# Autodesk Inventor assembly: NMR Frame
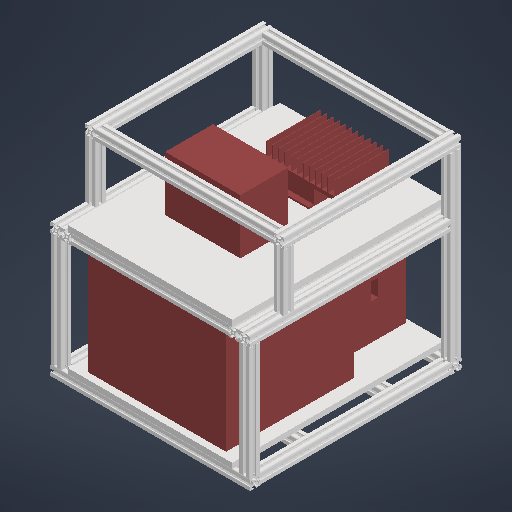
[picture p0: Inventor's stored thumbnail of the model, 512x512]
Saved by Autodesk Inventor 2026.2 (Build 302298010, 298A)
## iProperties
Created: 2026-08-09
Part Number: NMR Frame
Document SubType Name: Assembly
Designer: aiden
Author: aiden
## Documents named in this file (15)
- D:\[GitHub]\flowthrough-water-quality-monitoring-system\system_development\Moultrie\v0.4.2\NMRtray\Frame\NMR Frame.iam
- D:\[GitHub]\flowthrough-water-quality-monitoring-system\system_development\Moultrie\v0.4.2\NMRtray\Al Bars\AL369.575_5537T104.ipt
- D:\[GitHub]\flowthrough-water-quality-monitoring-system\system_development\Moultrie\v0.4.2\NMRtray\Al Bars\AL210_5537T104.ipt
- D:\[GitHub]\flowthrough-water-quality-monitoring-system\system_development\Moultrie\v0.4.2\NMRtray\Al Bars\AL336_5537T104.ipt
- D:\[GitHub]\flowthrough-water-quality-monitoring-system\system_development\Moultrie\v0.4.2\NMRtray\Al Bars\AL329.575_5537T104.ipt
- D:\[GitHub]\flowthrough-water-quality-monitoring-system\system_development\Moultrie\v0.4.2\NMRtray\Al Bars\AL106_5537T104.ipt
- D:\[GitHub]\flowthrough-water-quality-monitoring-system\system_development\Moultrie\v0.4.2\NMRtray\Al Bars\AL373.7_5537T104.ipt
- D:\[GitHub]\flowthrough-water-quality-monitoring-system\system_development\Moultrie\v0.4.2\NMRtray\Al Bars\AL393.7_5537T104.ipt
- D:\[GitHub]\flowthrough-water-quality-monitoring-system\system_development\Moultrie\v0.4.2\NMRtray\Al Bars\AL289.575_5537T104.ipt
- D:\[GitHub]\flowthrough-water-quality-monitoring-system\system_development\Moultrie\v0.4.2\NMRtray\Shelf.ipt
- D:\[GitHub]\flowthrough-water-quality-monitoring-system\system_development\Moultrie\v0.4.2\NMRtray\Electrical Components\Magnet.ipt
- D:\[GitHub]\flowthrough-water-quality-monitoring-system\system_development\Moultrie\v0.4.2\NMRtray\Electrical Components\Heatsink and Amplifier.ipt
- D:\[GitHub]\flowthrough-water-quality-monitoring-system\system_development\Moultrie\v0.4.2\NMRtray\Electrical Components\NMR Control Circuit Board.ipt
- D:\[GitHub]\flowthrough-water-quality-monitoring-system\system_development\Moultrie\v0.4.2\NMRtray\Electrical Components\NI PXIe_1071.ipt
- D:\[GitHub]\flowthrough-water-quality-monitoring-system\system_development\Moultrie\v0.4.2\NMRtray\Al Bars\AL353.7_5537T104.ipt
## Components (29 placed, 14 different names)
1. AL369.575_5537T104:1 — Rigid:4, Rigid:5, Flush:32, Mate:41, Mate:53
2. AL369.575_5537T104:2 — Rigid:6, Rigid:7, Mate:47, Flush:33, Flush:34, Mate:48, Flush:35, Flush:36, Mate:51
3. AL210_5537T104:1 — Rigid:5, Mate:21, Flush:8, Flush:26, Mate:42
4. AL210_5537T104:2 — Rigid:4, Mate:19, Flush:7, Flush:25
5. AL336_5537T104:1 — Rigid:6, Mate:10, Angle:3, Mate:18
6. AL336_5537T104:2 — Rigid:7, Mate:8, Angle:2, Mate:20, Angle:6, Flush:37, Mate:49
7. AL106_5537T104:1 — Mate:8, Mate:12, Angle:1, Flush:3, Mate:30, Flush:18, Mate:40
8. AL106_5537T104:2 — Mate:10, Mate:13, Flush:4, Mate:29, Flush:17
9. AL329.575_5537T104:2 — Mate:12, Angle:1, Flush:3, Angle:2, Flush:37, Mate:49
10. AL329.575_5537T104:3 — Mate:13, Flush:4, Angle:3, Mate:14, Angle:4, Flush:5, Mate:15, Flush:6, Angle:5
11. AL329.575_5537T104:4 — Mate:14, Angle:4, Flush:5
12. AL329.575_5537T104:5 — Mate:15, Flush:6, Angle:5
13. AL373.7_5537T104:1 — Mate:20, Mate:21, Flush:8, Mate:22, Flush:9, Flush:10, Mate:30, Flush:18, Flush:26, Mate:39
14. AL373.7_5537T104:2 — Mate:18, Mate:19, Flush:7, Mate:23, Flush:11, Flush:12, Mate:29, Flush:17, Flush:25
15. AL393.7_5537T104:1 — Mate:23, Flush:11, Flush:12
16. AL393.7_5537T104:2 — Mate:22, Flush:9, Flush:10, Mate:24, Flush:13, Flush:14, Mate:37, Flush:27, Flush:28, Mate:38, Flush:29, Flush:30
17. AL289.575_5537T104:1 — Mate:24, Flush:13, Flush:14
18. AL289.575_5537T104:4 — Mate:37, Flush:27, Flush:28, Flush:31
19. AL289.575_5537T104:5 — Mate:38, Flush:29, Flush:30
20. Shelf:1 — Flush:31, Mate:39, Mate:40, Mate:43, Mate:44
21. Shelf:2 — Flush:32, Mate:41, Mate:42, Mate:45, Mate:46
22. Magnet:1 — Mate:45, Angle:6
23. Heatsink and Amplifier:1 — Mate:43
24. NMR Control Circuit Board:1 — Mate:44
25. NI PXIe_1071:1 — Mate:46
26. AL353.7_5537T104:1 — Mate:48, Flush:35, Flush:36
27. AL353.7_5537T104:2 — Mate:47, Flush:33, Flush:34, Mate:50, Flush:38, Mate:52, Flush:39
28. AL329.575_5537T104:6 — Mate:50, Flush:38, Mate:51
29. AL329.575_5537T104:7 — Mate:52, Flush:39, Mate:53
## Relationships (71: Mate 32, Flush 29, Angle 6, WeldJoint 4)
- Rigid:4 [WeldJoint]: AL369.575_5537T104:1 ↔ AL210_5537T104:2
- Rigid:5 [WeldJoint]: AL369.575_5537T104:1 ↔ AL210_5537T104:1
- Rigid:6 [WeldJoint]: AL369.575_5537T104:2 ↔ AL336_5537T104:1
- Rigid:7 [WeldJoint]: AL369.575_5537T104:2 ↔ AL336_5537T104:2
- Mate:8 (290 mm): AL336_5537T104:2 ↔ AL106_5537T104:1
- Mate:10 (290 mm): AL336_5537T104:1 ↔ AL106_5537T104:2
- Mate:12: AL106_5537T104:1 ↔ AL329.575_5537T104:2
- Angle:1 (0 deg): AL106_5537T104:1 ↔ AL329.575_5537T104:2
- Flush:3: AL106_5537T104:1 ↔ AL329.575_5537T104:2
- Angle:2 (0 deg): AL336_5537T104:2 ↔ AL329.575_5537T104:2
- Mate:13: AL106_5537T104:2 ↔ AL329.575_5537T104:3
- Flush:4: AL106_5537T104:2 ↔ AL329.575_5537T104:3
- Angle:3 (0 deg): AL336_5537T104:1 ↔ AL329.575_5537T104:3
- Mate:14: AL329.575_5537T104:3 ↔ AL329.575_5537T104:4
- Angle:4 (90 deg): AL329.575_5537T104:3 ↔ AL329.575_5537T104:4
- Flush:5: AL329.575_5537T104:3 ↔ AL329.575_5537T104:4
- Mate:15: AL329.575_5537T104:3 ↔ AL329.575_5537T104:5
- Flush:6: AL329.575_5537T104:3 ↔ AL329.575_5537T104:5
- Angle:5 (90 deg): AL329.575_5537T104:3 ↔ AL329.575_5537T104:5
- Mate:18: AL336_5537T104:1 ↔ AL373.7_5537T104:2
- Mate:19: AL210_5537T104:2 ↔ AL373.7_5537T104:2
- Flush:7: AL210_5537T104:2 ↔ AL373.7_5537T104:2
- Mate:20: AL336_5537T104:2 ↔ AL373.7_5537T104:1
- Mate:21: AL210_5537T104:1 ↔ AL373.7_5537T104:1
- Flush:8: AL210_5537T104:1 ↔ AL373.7_5537T104:1
- Mate:22: AL373.7_5537T104:1 ↔ AL393.7_5537T104:2
- Flush:9: AL373.7_5537T104:1 ↔ AL393.7_5537T104:2
- Flush:10: AL373.7_5537T104:1 ↔ AL393.7_5537T104:2
- Mate:23: AL373.7_5537T104:2 ↔ AL393.7_5537T104:1
- Flush:11: AL373.7_5537T104:2 ↔ AL393.7_5537T104:1
- Flush:12: AL373.7_5537T104:2 ↔ AL393.7_5537T104:1
- Mate:24 (10 mm): AL393.7_5537T104:2 ↔ AL289.575_5537T104:1
- Flush:13: AL393.7_5537T104:2 ↔ AL289.575_5537T104:1
- Flush:14 (-196.85 mm): AL393.7_5537T104:2 ↔ AL289.575_5537T104:1
- Mate:29: AL106_5537T104:2 ↔ AL373.7_5537T104:2
- Flush:17: AL106_5537T104:2 ↔ AL373.7_5537T104:2
- Mate:30: AL106_5537T104:1 ↔ AL373.7_5537T104:1
- Flush:18: AL106_5537T104:1 ↔ AL373.7_5537T104:1
- Flush:25: AL210_5537T104:2 ↔ AL373.7_5537T104:2
- Flush:26: AL210_5537T104:1 ↔ AL373.7_5537T104:1
- Mate:37: AL393.7_5537T104:2 ↔ AL289.575_5537T104:4
- Flush:27: AL393.7_5537T104:2 ↔ AL289.575_5537T104:4
- Flush:28: AL393.7_5537T104:2 ↔ AL289.575_5537T104:4
- Mate:38: AL393.7_5537T104:2 ↔ AL289.575_5537T104:5
- Flush:29: AL393.7_5537T104:2 ↔ AL289.575_5537T104:5
- Flush:30: AL393.7_5537T104:2 ↔ AL289.575_5537T104:5
- Flush:31: AL289.575_5537T104:4 ↔ Shelf:1
- Mate:39: AL373.7_5537T104:1 ↔ Shelf:1
- Mate:40 (12.5 mm): AL106_5537T104:1 ↔ Shelf:1
- Flush:32: AL369.575_5537T104:1 ↔ Shelf:2
- Mate:41: AL369.575_5537T104:1 ↔ Shelf:2
- Mate:42 (12.5 mm): AL210_5537T104:1 ↔ Shelf:2
- Mate:43: Shelf:1 ↔ Heatsink and Amplifier:1
- Mate:44: Shelf:1 ↔ NMR Control Circuit Board:1
- Mate:45: Shelf:2 ↔ Magnet:1
- Mate:46: Shelf:2 ↔ NI PXIe_1071:1
- Angle:6 (90 deg): AL336_5537T104:2 ↔ Magnet:1
- Mate:47: AL369.575_5537T104:2 ↔ AL353.7_5537T104:2
- Flush:33: AL369.575_5537T104:2 ↔ AL353.7_5537T104:2
- Flush:34: AL369.575_5537T104:2 ↔ AL353.7_5537T104:2
- Mate:48: AL369.575_5537T104:2 ↔ AL353.7_5537T104:1
- Flush:35: AL369.575_5537T104:2 ↔ AL353.7_5537T104:1
- Flush:36: AL369.575_5537T104:2 ↔ AL353.7_5537T104:1
- Flush:37: AL336_5537T104:2 ↔ AL329.575_5537T104:2
- Mate:49: AL336_5537T104:2 ↔ AL329.575_5537T104:2
- Mate:50: AL353.7_5537T104:2 ↔ AL329.575_5537T104:6
- Flush:38: AL353.7_5537T104:2 ↔ AL329.575_5537T104:6
- Mate:51 (88.425 mm): AL369.575_5537T104:2 ↔ AL329.575_5537T104:6
- Mate:52: AL353.7_5537T104:2 ↔ AL329.575_5537T104:7
- Flush:39: AL353.7_5537T104:2 ↔ AL329.575_5537T104:7
- Mate:53 (88.425 mm): AL369.575_5537T104:1 ↔ AL329.575_5537T104:7
